# Autodesk Inventor assembly: Assembly1
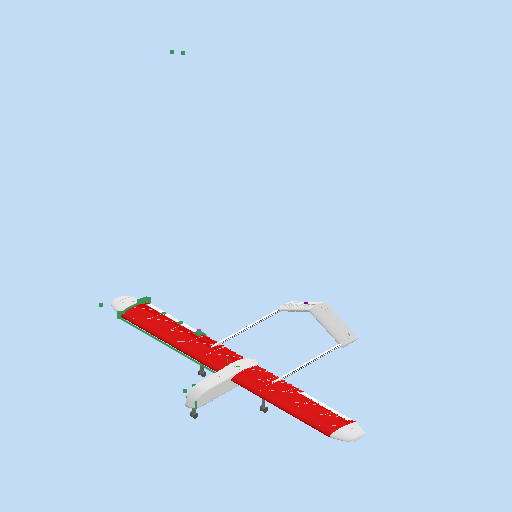
[picture p0: Inventor's stored thumbnail of the model, 512x512]
Saved by Autodesk Inventor 2026.1 (Build 301233000, 233)
## iProperties
Created: 2026-03-26
Part Number: Assembly1
Document SubType Name: Assembly
Designer: mateo
Author: mateo
## Documents named in this file (12)
- C:\GitHub\Senior-Design-UAV\Elytra CAD\Assembly\Assembly1.iam
- C:\GitHub\Senior-Design-UAV\Elytra CAD\Parts\Fueselage.ipt
- C:\GitHub\Senior-Design-UAV\Elytra CAD\20x20 Extrusions\20x20x2900ExtrudedAluminum.ipt
- C:\GitHub\Senior-Design-UAV\Elytra CAD\Parts\Cover.ipt
- C:\GitHub\Senior-Design-UAV\Elytra CAD\Parts\WingLeft2.ipt
- C:\GitHub\Senior-Design-UAV\Elytra CAD\Parts\WingMirror.ipt
- C:\GitHub\Senior-Design-UAV\Elytra CAD\Parts\Landing Gear\V2\LandingGearNose2.iam
- C:\GitHub\Senior-Design-UAV\Elytra CAD\20x20 Extrusions\20x20x800ExtrudedAluminum.ipt
- C:\GitHub\Senior-Design-UAV\Elytra CAD\Assembly\TailwAilerons.iam
- C:\GitHub\Senior-Design-UAV\Elytra CAD\Parts\Ailerons\AlerionLeft.ipt
- C:\GitHub\Senior-Design-UAV\Elytra CAD\Parts\Ailerons\AlerionLeft_MIR1.ipt
- C:\GitHub\Senior-Design-UAV\Elytra CAD\Parts\Landing Gear\V2\WingGear.iam
## Components (13 placed, 11 different names)
1. Fueselage:2 — Mate:1, Mate:2, Mate:3, Mate:4, Mate:6, Mate:7, Mate:10, Mate:17
2. 20x20x2900ExtrudedAluminum:1 — Mate:3, Mate:4, Mate:7, Mate:8, Mate:9, Mate:13, Mate:15, Mate:16
3. Cover:1 — Mate:5, Mate:6
4. WingLeft2:1 — Mate:9, Mate:10, Mate:12, Mate:19
5. WingMirror:1 — Mate:8, Mate:14, Mate:16, Mate:17
6. LandingGearNose2:1 [sub-assembly]
7. 20x20x800ExtrudedAluminum:1 — Mate:12, Mate:13
8. 20x20x800ExtrudedAluminum:2 — Mate:14, Mate:15, Mate:18
9. TailwAilerons:1 [sub-assembly] — Mate:18
10. AlerionLeft:1 — Mate:19
11. AlerionLeft_MIR1:1
12. WingGear:1 [sub-assembly]
13. WingGear:2 [sub-assembly]
## Relationships (18: Mate 18)
- Mate:1: Fueselage:2
- Mate:2: Fueselage:2
- Mate:3: Fueselage:2 ↔ 20x20x2900ExtrudedAluminum:1
- Mate:4: Fueselage:2 ↔ 20x20x2900ExtrudedAluminum:1
- Mate:5: Cover:1
- Mate:6: Fueselage:2 ↔ Cover:1
- Mate:7: Fueselage:2 ↔ 20x20x2900ExtrudedAluminum:1
- Mate:8: 20x20x2900ExtrudedAluminum:1 ↔ WingMirror:1
- Mate:9: 20x20x2900ExtrudedAluminum:1 ↔ WingLeft2:1
- Mate:10: Fueselage:2 ↔ WingLeft2:1
- Mate:12: WingLeft2:1 ↔ 20x20x800ExtrudedAluminum:1
- Mate:13: 20x20x2900ExtrudedAluminum:1 ↔ 20x20x800ExtrudedAluminum:1
- Mate:14: WingMirror:1 ↔ 20x20x800ExtrudedAluminum:2
- Mate:15: 20x20x2900ExtrudedAluminum:1 ↔ 20x20x800ExtrudedAluminum:2
- Mate:16: 20x20x2900ExtrudedAluminum:1 ↔ WingMirror:1
- Mate:17: Fueselage:2 ↔ WingMirror:1
- Mate:18: 20x20x800ExtrudedAluminum:2 ↔ TailwAilerons:1
- Mate:19: WingLeft2:1 ↔ AlerionLeft:1
